# Autodesk Inventor assembly: 垃圾桶上层
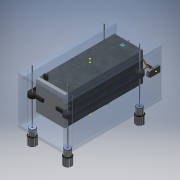
[picture p0: Inventor's stored thumbnail of the model, 180x180]
Saved by Autodesk Inventor 2017 (Build 210142000, 142)
## iProperties
Part Number: 垃圾桶上层
Material: 常规
Document SubType Name: Assembly
Designer: PANDA
Author: PANDA
## Documents named in this file (16)
- D:\PANDA\Study\VG100\P2\草图\垃圾桶上层.iam
- D:\PANDA\Study\VG100\P2\草图\垃圾桶正版.ipt
- D:\PANDA\Study\VG100\P2\草图\垃圾桶侧板.ipt
- D:\PANDA\Study\VG100\P2\草图\马达.ipt
- D:\PANDA\Study\VG100\P2\草图\姿态传感器.ipt
- D:\PANDA\Study\VG100\P2\草图\激光传感器.ipt
- D:\PANDA\Study\VG100\P2\草图\长轴.ipt
- D:\PANDA\Study\VG100\P2\草图\皮带轮.ipt
- D:\PANDA\Study\VG100\P2\草图\皮带.ipt
- D:\PANDA\Study\VG100\P2\草图\升降板.ipt
- D:\PANDA\Study\VG100\P2\草图\内层升降板.ipt
- D:\PANDA\Study\VG100\P2\草图\内层正板.ipt
- D:\PANDA\Study\VG100\P2\草图\内层侧板.ipt
- D:\PANDA\Study\VG100\P2\草图\推杆电机.ipt
- D:\PANDA\Study\VG100\P2\草图\打包支架.ipt
- D:\PANDA\Study\VG100\P2\草图\压缩杆.ipt
## Components (34 placed, 15 different names)
1. 垃圾桶正版:1 — 旋转:3, 旋转:7
2. 垃圾桶侧板:2 — 旋转:3, 旋转:4, 旋转:5, 刚性:22
3. 垃圾桶正版:2 — 旋转:4, 旋转:5, 旋转:6, 旋转:32, 旋转:33, 旋转:49, 旋转:50
4. 垃圾桶侧板:3 — 旋转:6, 旋转:7, 旋转:58
5. 马达:5 — 旋转:33, 旋转:39
6. 马达:7 — 旋转:32, 旋转:36
7. 长轴:2 — 旋转:36, 刚性:8
8. 皮带轮:2 — 刚性:8, 旋转:54
9. 长轴:5 — 旋转:39, 刚性:10
10. 皮带轮:8 — 刚性:10, 旋转:56
11. 升降板:1
12. 升降板:2 — 刚性:17
13. 内层升降板:1 — 刚性:17, 旋转:44, 旋转:45, 旋转:46, 旋转:47, 旋转:48
14. 内层正板:1 — 旋转:44, 旋转:57
15. 内层正板:2 — 旋转:45, 刚性:20
16. 内层侧板:1 — 旋转:46
17. 内层侧板:2 — 旋转:47, 旋转:48
18. 马达:9 — 旋转:49, 旋转:51
19. 长轴:6 — 旋转:52, 刚性:18
20. 长轴:7 — 旋转:51, 刚性:19
21. 马达:10 — 旋转:50, 旋转:52
22. 皮带轮:9 — 刚性:19, 旋转:53
23. 皮带轮:10 — 刚性:18, 旋转:55
24. 皮带:1 — 旋转:53, 旋转:54
25. 皮带:2 — 旋转:55, 旋转:56
26. 激光传感器:3 — 刚性:20
27. 激光传感器:4 — 旋转:57
28. 姿态传感器:1
29. 推杆电机:1 — 旋转:58, 旋转:60
30. 打包支架:1 — 旋转:59, 旋转:62
31. 打包支架:2 — 旋转:60, 旋转:61
32. 推杆电机:2 — 刚性:22, 旋转:59
33. 压缩杆:1 — 旋转:61
34. 压缩杆:2 — 旋转:62
## Relationships (35: RevoluteJoint 28, WeldJoint 7)
- 旋转:3 [RevoluteJoint]: 垃圾桶正版:1 ↔ 垃圾桶侧板:2
- 旋转:4 [RevoluteJoint]: 垃圾桶侧板:2 ↔ 垃圾桶正版:2
- 旋转:5 [RevoluteJoint]: 垃圾桶侧板:2 ↔ 垃圾桶正版:2
- 旋转:6 [RevoluteJoint]: 垃圾桶正版:2 ↔ 垃圾桶侧板:3
- 旋转:7 [RevoluteJoint]: 垃圾桶正版:1 ↔ 垃圾桶侧板:3
- 旋转:32 [RevoluteJoint]: 垃圾桶正版:2 ↔ 马达:7
- 旋转:33 [RevoluteJoint]: 垃圾桶正版:2 ↔ 马达:5
- 旋转:36 [RevoluteJoint]: 马达:7 ↔ 长轴:2
- 刚性:8 [WeldJoint]: 长轴:2 ↔ 皮带轮:2
- 旋转:39 [RevoluteJoint]: 马达:5 ↔ 长轴:5
- 刚性:10 [WeldJoint]: 长轴:5 ↔ 皮带轮:8
- 刚性:17 [WeldJoint]: 升降板:2 ↔ 内层升降板:1
- 旋转:44 [RevoluteJoint]: 内层升降板:1 ↔ 内层正板:1
- 旋转:45 [RevoluteJoint]: 内层升降板:1 ↔ 内层正板:2
- 旋转:46 [RevoluteJoint]: 内层升降板:1 ↔ 内层侧板:1
- 旋转:47 [RevoluteJoint]: 内层升降板:1 ↔ 内层侧板:2
- 旋转:48 [RevoluteJoint]: 内层升降板:1 ↔ 内层侧板:2
- 旋转:49 [RevoluteJoint]: 垃圾桶正版:2 ↔ 马达:9
- 旋转:50 [RevoluteJoint]: 垃圾桶正版:2 ↔ 马达:10
- 旋转:51 [RevoluteJoint]: 马达:9 ↔ 长轴:7
- 旋转:52 [RevoluteJoint]: 长轴:6 ↔ 马达:10
- 刚性:18 [WeldJoint]: 长轴:6 ↔ 皮带轮:10
- 刚性:19 [WeldJoint]: 长轴:7 ↔ 皮带轮:9
- 旋转:53 [RevoluteJoint]: 皮带轮:9 ↔ 皮带:1
- 旋转:54 [RevoluteJoint]: 皮带轮:2 ↔ 皮带:1
- 旋转:55 [RevoluteJoint]: 皮带轮:10 ↔ 皮带:2
- 旋转:56 [RevoluteJoint]: 皮带轮:8 ↔ 皮带:2
- 刚性:20 [WeldJoint]: 内层正板:2 ↔ 激光传感器:3
- 旋转:57 [RevoluteJoint]: 内层正板:1 ↔ 激光传感器:4
- 旋转:58 [RevoluteJoint]: 垃圾桶侧板:3 ↔ 推杆电机:1
- 刚性:22 [WeldJoint]: 垃圾桶侧板:2 ↔ 推杆电机:2
- 旋转:59 [RevoluteJoint]: 打包支架:1 ↔ 推杆电机:2
- 旋转:60 [RevoluteJoint]: 推杆电机:1 ↔ 打包支架:2
- 旋转:61 [RevoluteJoint]: 打包支架:2 ↔ 压缩杆:1
- 旋转:62 [RevoluteJoint]: 打包支架:1 ↔ 压缩杆:2
